# Autodesk Inventor assembly: Sheathing_For_Front
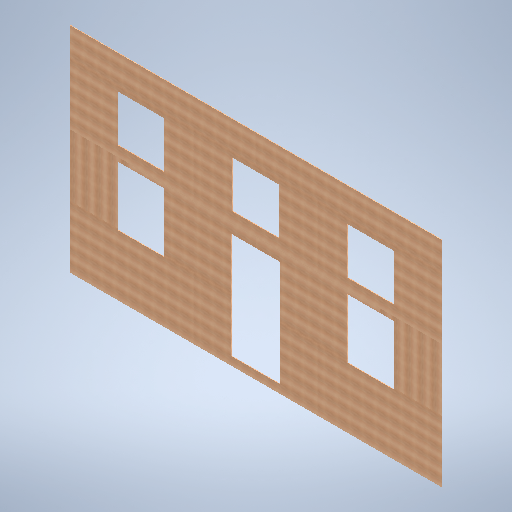
[picture p0: Inventor's stored thumbnail of the model, 512x512]
Saved by Autodesk Inventor 2025.1 (Build 291241020, 241B)
## iProperties
Created: 2024-10-03
Part Number: Sheathing_For_Front
Document SubType Name: Assembly
Designer: Tom
Author: Tom
## Documents named in this file (5)
- C:\Users\Tom\Documents\Inventor\Mobility\Additional_Building\Sheathing_For_Front.iam
- C:\Users\Tom\Documents\Inventor\Mobility\Additional_Building\OSB_For_Walls_With_Dimensions_48_x_96_Inches.ipt
- C:\Users\Tom\Documents\Inventor\Mobility\Additional_Building\OSB_For_Walls_With_Dimensions_48_x_48_Inches.ipt
- C:\Users\Tom\Documents\Inventor\Mobility\Additional_Building\OSB_For_Walls_With_Dimensions_21.796_x_48_Inches.ipt
- C:\Users\Tom\Documents\Inventor\Mobility\Additional_Building\OSB_For_Walls_With_Dimensions_21.796_x_96_Inches.ipt
## Components (14 placed, 4 different names)
1. OSB_For_Walls_With_Dimensions_48_x_96_Inches:1 — Mate:1, Mate:2, Flush:1, Mate:3, Flush:2, Flush:3, Flush:4
2. OSB_For_Walls_With_Dimensions_48_x_96_Inches:2 — Mate:4
3. OSB_For_Walls_With_Dimensions_48_x_96_Inches:3
4. OSB_For_Walls_With_Dimensions_48_x_96_Inches:4 — Mate:4, Mate:5, Flush:4
5. OSB_For_Walls_With_Dimensions_48_x_96_Inches:5
6. OSB_For_Walls_With_Dimensions_48_x_48_Inches:1 — Mate:3, Flush:2, Flush:3, Mate:5, Mate:6, Flush:5, Flush:6
7. OSB_For_Walls_With_Dimensions_48_x_48_Inches:2
8. OSB_For_Walls_With_Dimensions_48_x_96_Inches:6 — Mate:6, Flush:5, Flush:6, Mate:7, Flush:7, Flush:8, Mate:8
9. OSB_For_Walls_With_Dimensions_48_x_96_Inches:7
10. OSB_For_Walls_With_Dimensions_48_x_96_Inches:8
11. OSB_For_Walls_With_Dimensions_21.796_x_96_Inches:1 — Mate:8, Mate:9, Flush:9
12. OSB_For_Walls_With_Dimensions_21.796_x_96_Inches:2
13. OSB_For_Walls_With_Dimensions_21.796_x_48_Inches:1 — Mate:7, Flush:7, Flush:8, Mate:9, Flush:9
14. OSB_For_Walls_With_Dimensions_21.796_x_48_Inches:2
## Component patterns: (3 elements, first: OSB_For_Walls_With_Dimensions_48_x_96_Inches:1), (2 elements, first: OSB_For_Walls_With_Dimensions_48_x_96_Inches:4), (2 elements, first: OSB_For_Walls_With_Dimensions_48_x_48_Inches:1), (3 elements, first: OSB_For_Walls_With_Dimensions_48_x_96_Inches:6), (2 elements, first: OSB_For_Walls_With_Dimensions_21.796_x_96_Inches:1), (2 elements, first: OSB_For_Walls_With_Dimensions_21.796_x_48_Inches:1)
## Relationships (18: Mate 9, Flush 9)
- Mate:1: OSB_For_Walls_With_Dimensions_48_x_96_Inches:1
- Mate:2: OSB_For_Walls_With_Dimensions_48_x_96_Inches:1
- Flush:1: OSB_For_Walls_With_Dimensions_48_x_96_Inches:1
- Mate:3: OSB_For_Walls_With_Dimensions_48_x_96_Inches:1 ↔ OSB_For_Walls_With_Dimensions_48_x_48_Inches:1
- Flush:2: OSB_For_Walls_With_Dimensions_48_x_96_Inches:1 ↔ OSB_For_Walls_With_Dimensions_48_x_48_Inches:1
- Flush:3: OSB_For_Walls_With_Dimensions_48_x_96_Inches:1 ↔ OSB_For_Walls_With_Dimensions_48_x_48_Inches:1
- Mate:4: OSB_For_Walls_With_Dimensions_48_x_96_Inches:2 ↔ OSB_For_Walls_With_Dimensions_48_x_96_Inches:4
- Mate:5: OSB_For_Walls_With_Dimensions_48_x_96_Inches:4 ↔ OSB_For_Walls_With_Dimensions_48_x_48_Inches:1
- Flush:4: OSB_For_Walls_With_Dimensions_48_x_96_Inches:1 ↔ OSB_For_Walls_With_Dimensions_48_x_96_Inches:4
- Mate:6: OSB_For_Walls_With_Dimensions_48_x_48_Inches:1 ↔ OSB_For_Walls_With_Dimensions_48_x_96_Inches:6
- Flush:5: OSB_For_Walls_With_Dimensions_48_x_48_Inches:1 ↔ OSB_For_Walls_With_Dimensions_48_x_96_Inches:6
- Flush:6: OSB_For_Walls_With_Dimensions_48_x_48_Inches:1 ↔ OSB_For_Walls_With_Dimensions_48_x_96_Inches:6
- Mate:7: OSB_For_Walls_With_Dimensions_48_x_96_Inches:6 ↔ OSB_For_Walls_With_Dimensions_21.796_x_48_Inches:1
- Flush:7: OSB_For_Walls_With_Dimensions_48_x_96_Inches:6 ↔ OSB_For_Walls_With_Dimensions_21.796_x_48_Inches:1
- Flush:8: OSB_For_Walls_With_Dimensions_48_x_96_Inches:6 ↔ OSB_For_Walls_With_Dimensions_21.796_x_48_Inches:1
- Mate:8: OSB_For_Walls_With_Dimensions_48_x_96_Inches:6 ↔ OSB_For_Walls_With_Dimensions_21.796_x_96_Inches:1
- Mate:9: OSB_For_Walls_With_Dimensions_21.796_x_96_Inches:1 ↔ OSB_For_Walls_With_Dimensions_21.796_x_48_Inches:1
- Flush:9: OSB_For_Walls_With_Dimensions_21.796_x_96_Inches:1 ↔ OSB_For_Walls_With_Dimensions_21.796_x_48_Inches:1
